# Autodesk Inventor assembly: hatch above arm
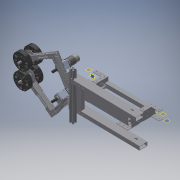
[picture p0: Inventor's stored thumbnail of the model, 180x180]
Saved by Autodesk Inventor 2018 (Build 220112000, 112)
## iProperties
Created: 2019-01-20
Part Number: hatch above arm
Document SubType Name: Assembly
Designer: Burni
Author: Burni
## Documents named in this file (10)
- C:\Users\s-4008082\Downloads\2019CAD-master\2019CAD-master\Hatch design with heightened hatch\hatch above arm.iam
- C:\Users\s-4008082\Downloads\2019CAD-master\2019CAD-master\Hatch design with heightened hatch\left arm.ipt
- C:\Users\s-4008082\Downloads\2019CAD-master\2019CAD-master\Hatch design with heightened hatch\right arm.ipt
- C:\Users\s-4008082\Downloads\2019CAD-master\2019CAD-master\Hatch design with heightened hatch\push bar.ipt
- C:\Users\s-4008082\Downloads\2019CAD-master\2019CAD-master\Hatch design with heightened hatch\PARTserver02019011803125824465437192d056f\AIS2018\021-DXP(F,D-770).iam
- C:\Users\s-4008082\Downloads\2019CAD-master\2019CAD-master\Hatch design with heightened hatch\Bracing 3x3.ipt
- C:\Users\s-4008082\Downloads\2019CAD-master\2019CAD-master\Hatch design with heightened hatch\ATACHMENT BAR.ipt
- C:\Users\s-4008082\Downloads\2019CAD-master\2019CAD-master\Hatch design with heightened hatch\Mounting part.ipt
- C:\Users\s-4008082\Downloads\2019CAD-master\2019CAD-master\Hatch design with heightened hatch\mounting part 2.ipt
- C:\Users\s-4008082\Downloads\2019CAD-master  DELETE OTHERS(4)\2019CAD-master\Ball Intake ver 2\MAIN Gripper assembly.iam
## Components (18 placed, 9 different names)
1. left arm:1 — Flush:32, Flush:34, Mate:19, Flush:35, Mate:20, Flush:37, Mate:25, Mate:26
2. right arm:1 — Flush:32, Flush:33, Mate:22, Flush:38
3. push bar:1
4. 021-DXP(F,D-770):1 [sub-assembly]
5. 021-DXP(F,D-770):2 [sub-assembly] — Flush:33
6. Bracing 3x3:1
7. Bracing 3x3:2
8. Bracing 3x3:3
9. Bracing 3x3:4
10. Bracing 3x3:5 — Mate:25, Mate:26, Mate:27, Mate:28
11. Bracing 3x3:6 — Mate:21, Mate:22, Mate:23
12. Bracing 3x3:7 — Mate:29, Flush:38, Mate:30
13. Bracing 3x3:8 — Mate:20, Flush:37, Mate:24
14. ATACHMENT BAR:1 — Flush:34, Mate:19, Flush:35, Mate:21, Mate:23, Mate:24, Mate:27, Mate:28, Mate:29, Mate:30, Mate:31, Mate:32, Flush:44
15. Mounting part:1 — Mate:31, Mate:32, Flush:39, Mate:34, Mate:35, Flush:40, Flush:41, Mate:36, Flush:43, Flush:44, Mate:37
16. mounting part 2:1 — Flush:39, Mate:34, Mate:36, Flush:42
17. mounting part 2:2 — Mate:35, Flush:40, Flush:41
18. MAIN Gripper assembly:1 [sub-assembly] — Flush:42, Flush:43, Mate:37
## Relationships (52: Mate 29, Flush 23)
- [Mate]: left arm:1 ↔ 021-DXP(F,D-770):1
- [Mate]: right arm:1 ↔ 021-DXP(F,D-770):2
- [Flush]: right arm:1 ↔ Bracing 3x3:4
- [Flush]: right arm:1 ↔ Bracing 3x3:4
- [Mate]: right arm:1 ↔ Bracing 3x3:4
- [Flush]: right arm:1 ↔ Bracing 3x3:3
- [Mate]: right arm:1 ↔ Bracing 3x3:3
- [Flush]: right arm:1 ↔ Bracing 3x3:3
- [Flush]: left arm:1 ↔ Bracing 3x3:1
- [Flush]: left arm:1 ↔ Bracing 3x3:1
- [Mate]: left arm:1 ↔ Bracing 3x3:1
- [Mate]: left arm:1 ↔ Bracing 3x3:2
- [Flush]: left arm:1 ↔ Bracing 3x3:2
- [Flush]: left arm:1 ↔ Bracing 3x3:2
- [Flush]: left arm:1 ↔ right arm:1
- [Mate] (2.54 mm): push bar:1 ↔ 021-DXP(F,D-770):2
- [Mate] (279.4 mm): left arm:1 ↔ right arm:1
- [Mate]: push bar:1 ↔ 021-DXP(F,D-770):2
- [Mate] (2.54 mm): push bar:1 ↔ 021-DXP(F,D-770):1
- [Mate]: push bar:1 ↔ 021-DXP(F,D-770):1
- [Flush] (38.1 mm): right arm:1 ↔ 021-DXP(F,D-770):2
- [Flush] (38.1 mm): left arm:1 ↔ 021-DXP(F,D-770):1
- Flush:32: left arm:1 ↔ right arm:1
- Flush:33 (11.938 mm): right arm:1 ↔ 021-DXP(F,D-770):2
- Flush:34: left arm:1 ↔ ATACHMENT BAR:1
- Mate:19: left arm:1 ↔ ATACHMENT BAR:1
- Flush:35: left arm:1 ↔ ATACHMENT BAR:1
- Mate:20: left arm:1 ↔ Bracing 3x3:8
- Mate:21: Bracing 3x3:6 ↔ ATACHMENT BAR:1
- Mate:22: right arm:1 ↔ Bracing 3x3:6
- Flush:37: left arm:1 ↔ Bracing 3x3:8
- Mate:23: Bracing 3x3:6 ↔ ATACHMENT BAR:1
- Mate:24: Bracing 3x3:8 ↔ ATACHMENT BAR:1
- Mate:25: left arm:1 ↔ Bracing 3x3:5
- Mate:26: left arm:1 ↔ Bracing 3x3:5
- Mate:27: Bracing 3x3:5 ↔ ATACHMENT BAR:1
- Mate:28: Bracing 3x3:5 ↔ ATACHMENT BAR:1
- Mate:29: Bracing 3x3:7 ↔ ATACHMENT BAR:1
- Flush:38: right arm:1 ↔ Bracing 3x3:7
- Mate:30: Bracing 3x3:7 ↔ ATACHMENT BAR:1
- Mate:31: ATACHMENT BAR:1 ↔ Mounting part:1
- Mate:32 (-101.6 mm): ATACHMENT BAR:1 ↔ Mounting part:1
- Flush:39: Mounting part:1 ↔ mounting part 2:1
- Mate:34: Mounting part:1 ↔ mounting part 2:1
- Mate:35: Mounting part:1 ↔ mounting part 2:2
- Flush:40: Mounting part:1 ↔ mounting part 2:2
- Flush:41: Mounting part:1 ↔ mounting part 2:2
- Mate:36: Mounting part:1 ↔ mounting part 2:1
- Flush:42 (-50.8 mm): mounting part 2:1 ↔ MAIN Gripper assembly:1
- Flush:43: Mounting part:1 ↔ MAIN Gripper assembly:1
- Flush:44: ATACHMENT BAR:1 ↔ Mounting part:1
- Mate:37: Mounting part:1 ↔ MAIN Gripper assembly:1
## Named parameters: d9_d32 = 0 mm
